# Autodesk Inventor assembly: Ensamblaje carcasa
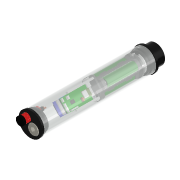
[picture p0: Inventor's stored thumbnail of the model, 180x180]
Saved by Autodesk Inventor 2022.3 (Build 263350000, 350)
## iProperties
Created: 2023-07-17
Part Number: Ensamblaje carcasa
Document SubType Name: Assembly
Designer: Usuario
Author: Usuario
## Documents named in this file (20)
- C:\Users\Usuario\OneDrive - Universidad de Salamanca\Universidad - Doctorado\Estancia Extranjero\3. Desarrollo e Investigación\Bouy enclosure\Ensamblaje carcasa - v2.iam
- C:\Users\Usuario\OneDrive - Universidad de Salamanca\Universidad - Doctorado\Estancia Extranjero\3. Desarrollo e Investigación\Bouy enclosure\Cilindro_hueco.ipt
- C:\Users\Usuario\OneDrive - Universidad de Salamanca\Universidad - Doctorado\Estancia Extranjero\3. Desarrollo e Investigación\Bouy enclosure\Junta_torica_pieza_sonar.ipt
- C:\Users\Usuario\OneDrive - Universidad de Salamanca\Universidad - Doctorado\Estancia Extranjero\3. Desarrollo e Investigación\Bouy enclosure\Junta_torica_sonar.ipt
- C:\Users\Usuario\OneDrive - Universidad de Salamanca\Universidad - Doctorado\Estancia Extranjero\3. Desarrollo e Investigación\Bouy enclosure\Pieza_sonar.ipt
- C:\Users\Usuario\OneDrive - Universidad de Salamanca\Universidad - Doctorado\Estancia Extranjero\3. Desarrollo e Investigación\Bouy enclosure\Sonar.ipt
- C:\Users\Usuario\OneDrive - Universidad de Salamanca\Universidad - Doctorado\Estancia Extranjero\3. Desarrollo e Investigación\Bouy enclosure\Pieza_conectores.ipt
- C:\Users\Usuario\OneDrive - Universidad de Salamanca\Universidad - Doctorado\Estancia Extranjero\3. Desarrollo e Investigación\Bouy enclosure\Cuerpo_interruptor_BlueRobotics.ipt
- C:\Users\Usuario\OneDrive - Universidad de Salamanca\Universidad - Doctorado\Estancia Extranjero\3. Desarrollo e Investigación\Bouy enclosure\Interruptor_BlueRobotics.ipt
- C:\Users\Usuario\OneDrive - Universidad de Salamanca\Universidad - Doctorado\Estancia Extranjero\3. Desarrollo e Investigación\Bouy enclosure\Tapon_interruptor_BlueRobotics.ipt
- C:\Users\Usuario\OneDrive - Universidad de Salamanca\Universidad - Doctorado\Estancia Extranjero\3. Desarrollo e Investigación\Bouy enclosure\Tuerca_interruptor_BlueRobotics.ipt
- C:\Users\Usuario\OneDrive - Universidad de Salamanca\Universidad - Doctorado\Estancia Extranjero\3. Desarrollo e Investigación\Bouy enclosure\Tuerca_pieza_conectores.ipt
- C:\Users\Usuario\OneDrive - Universidad de Salamanca\Universidad - Doctorado\Estancia Extranjero\3. Desarrollo e Investigación\Bouy enclosure\Sujección_piezas_sonar.ipt
- C:\Users\Usuario\OneDrive - Universidad de Salamanca\Universidad - Doctorado\Estancia Extranjero\3. Desarrollo e Investigación\Bouy enclosure\Sujección_Baterias.ipt
- C:\Users\Usuario\OneDrive - Universidad de Salamanca\Universidad - Doctorado\Estancia Extranjero\3. Desarrollo e Investigación\Bouy enclosure\Batería.ipt
- C:\Users\Usuario\OneDrive - Universidad de Salamanca\Universidad - Doctorado\Estancia Extranjero\3. Desarrollo e Investigación\Bouy enclosure\ESP32.ipt
- C:\Users\Usuario\OneDrive - Universidad de Salamanca\Universidad - Doctorado\Estancia Extranjero\3. Desarrollo e Investigación\Bouy enclosure\Nano-modem.ipt
- C:\Users\Usuario\OneDrive - Universidad de Salamanca\Universidad - Doctorado\Estancia Extranjero\3. Desarrollo e Investigación\Bouy enclosure\Nordic_PCB.ipt
- C:\Users\Usuario\OneDrive - Universidad de Salamanca\Universidad - Doctorado\Estancia Extranjero\3. Desarrollo e Investigación\Bouy enclosure\Sujeccion_PCBs - v2.ipt
- C:\Users\Usuario\OneDrive - Universidad de Salamanca\Universidad - Doctorado\Estancia Extranjero\3. Desarrollo e Investigación\Bouy enclosure\GPS.ipt
## Components (22 placed, 19 different names)
1. Cilindro_hueco:1 — Coincidencia:5, Coincidencia:6
2. Junta_torica_pieza_sonar:1 — Coincidencia:3
3. Junta_torica_sonar:1 — Coincidencia:1
4. Pieza_sonar:1 — Coincidencia:2, Coincidencia:3, Coincidencia:4, Coincidencia:5, Coincidencia:18, Coincidencia:23
5. Sonar:1 — Coincidencia:1, Coincidencia:2, Coincidencia:4
6. Pieza_conectores:1 — Coincidencia:6, Coincidencia:7, Ángulo:1, Coincidencia:11, Coincidencia:13, Coincidencia:15, Tangente:1, Tangente:2, Coincidencia:16, Coincidencia:17
7. Cuerpo_interruptor_BlueRobotics:1 — Coincidencia:7, Ángulo:1, Coincidencia:8, Coincidencia:9, Coincidencia:10, Coincidencia:11, Coincidencia:12, Coincidencia:14
8. Interruptor_BlueRobotics:1 — Coincidencia:10, Coincidencia:14
9. Tapon_interruptor_BlueRobotics:1 — Coincidencia:9, Coincidencia:12
10. Tuerca_interruptor_BlueRobotics:1 — Coincidencia:8, Coincidencia:13
11. Junta_torica_pieza_sonar:2 — Coincidencia:15, Tangente:1, Tangente:2
12. Tuerca_pieza_conectores:1 — Coincidencia:16, Coincidencia:17
13. Sujección_piezas_sonar:1 — Coincidencia:18, Coincidencia:19, Ángulo:2, Coincidencia:23, Coincidencia:24
14. Sujección_Baterias:1 — Coincidencia:19, Ángulo:2, Coincidencia:20, Coincidencia:21, Coincidencia:22, Coincidencia:24, Coincidencia:33, Coincidencia:34
15. Batería:1 — Coincidencia:20
16. Batería:2 — Coincidencia:22
17. Batería:3 — Coincidencia:21
18. ESP32:1 — Coincidencia:38, Coincidencia:39, Coincidencia:40
19. Nano-modem:1 — Coincidencia:31, Coincidencia:32, Coincidencia:35, Coincidencia:36, Coincidencia:37
20. Nordic_PCB:1 — Coincidencia:31, Coincidencia:32
21. Sujeccion_PCBs - v2:1 — Coincidencia:33, Coincidencia:34, Coincidencia:35, Coincidencia:36, Coincidencia:37, Coincidencia:38, Coincidencia:39, Coincidencia:40, Coincidencia:41, Coincidencia:42, Coincidencia:43
22. GPS:1 — Coincidencia:41, Coincidencia:42, Coincidencia:43
## Relationships (41: Mate 37, Angle 2, Tangent 2)
- Coincidencia:1 [Mate]: Junta_torica_sonar:1 ↔ Sonar:1
- Coincidencia:2 [Mate]: Pieza_sonar:1 ↔ Sonar:1
- Coincidencia:3 [Mate]: Junta_torica_pieza_sonar:1 ↔ Pieza_sonar:1
- Coincidencia:4 [Mate]: Pieza_sonar:1 ↔ Sonar:1
- Coincidencia:5 [Mate]: Cilindro_hueco:1 ↔ Pieza_sonar:1
- Coincidencia:6 [Mate]: Cilindro_hueco:1 ↔ Pieza_conectores:1
- Coincidencia:7 [Mate]: Pieza_conectores:1 ↔ Cuerpo_interruptor_BlueRobotics:1
- Ángulo:1 [Angle] (0 deg): Pieza_conectores:1 ↔ Cuerpo_interruptor_BlueRobotics:1
- Coincidencia:8 [Mate]: Cuerpo_interruptor_BlueRobotics:1 ↔ Tuerca_interruptor_BlueRobotics:1
- Coincidencia:9 [Mate]: Cuerpo_interruptor_BlueRobotics:1 ↔ Tapon_interruptor_BlueRobotics:1
- Coincidencia:10 [Mate]: Cuerpo_interruptor_BlueRobotics:1 ↔ Interruptor_BlueRobotics:1
- Coincidencia:11 [Mate]: Pieza_conectores:1 ↔ Cuerpo_interruptor_BlueRobotics:1
- Coincidencia:12 [Mate]: Cuerpo_interruptor_BlueRobotics:1 ↔ Tapon_interruptor_BlueRobotics:1
- Coincidencia:13 [Mate]: Pieza_conectores:1 ↔ Tuerca_interruptor_BlueRobotics:1
- Coincidencia:14 [Mate]: Cuerpo_interruptor_BlueRobotics:1 ↔ Interruptor_BlueRobotics:1
- Coincidencia:15 [Mate]: Pieza_conectores:1 ↔ Junta_torica_pieza_sonar:2
- Tangente:1: Pieza_conectores:1 ↔ Junta_torica_pieza_sonar:2
- Tangente:2: Pieza_conectores:1 ↔ Junta_torica_pieza_sonar:2
- Coincidencia:16 [Mate]: Pieza_conectores:1 ↔ Tuerca_pieza_conectores:1
- Coincidencia:17 [Mate]: Pieza_conectores:1 ↔ Tuerca_pieza_conectores:1
- Coincidencia:18 [Mate]: Pieza_sonar:1 ↔ Sujección_piezas_sonar:1
- Coincidencia:19 [Mate]: Sujección_piezas_sonar:1 ↔ Sujección_Baterias:1
- Ángulo:2 [Angle] (0 deg): Sujección_piezas_sonar:1 ↔ Sujección_Baterias:1
- Coincidencia:20 [Mate]: Sujección_Baterias:1 ↔ Batería:1
- Coincidencia:21 [Mate]: Sujección_Baterias:1 ↔ Batería:3
- Coincidencia:22 [Mate]: Sujección_Baterias:1 ↔ Batería:2
- Coincidencia:23 [Mate]: Pieza_sonar:1 ↔ Sujección_piezas_sonar:1
- Coincidencia:24 [Mate]: Sujección_piezas_sonar:1 ↔ Sujección_Baterias:1
- Coincidencia:31 [Mate]: Nano-modem:1 ↔ Nordic_PCB:1
- Coincidencia:32 [Mate]: Nano-modem:1 ↔ Nordic_PCB:1
- Coincidencia:33 [Mate]: Sujección_Baterias:1 ↔ Sujeccion_PCBs - v2:1
- Coincidencia:34 [Mate]: Sujección_Baterias:1 ↔ Sujeccion_PCBs - v2:1
- Coincidencia:35 [Mate]: Nano-modem:1 ↔ Sujeccion_PCBs - v2:1
- Coincidencia:36 [Mate]: Nano-modem:1 ↔ Sujeccion_PCBs - v2:1
- Coincidencia:37 [Mate]: Nano-modem:1 ↔ Sujeccion_PCBs - v2:1
- Coincidencia:38 [Mate]: ESP32:1 ↔ Sujeccion_PCBs - v2:1
- Coincidencia:39 [Mate]: ESP32:1 ↔ Sujeccion_PCBs - v2:1
- Coincidencia:40 [Mate]: ESP32:1 ↔ Sujeccion_PCBs - v2:1
- Coincidencia:41 [Mate]: Sujeccion_PCBs - v2:1 ↔ GPS:1
- Coincidencia:42 [Mate]: Sujeccion_PCBs - v2:1 ↔ GPS:1
- Coincidencia:43 [Mate]: Sujeccion_PCBs - v2:1 ↔ GPS:1
